# Autodesk Inventor assembly: 50
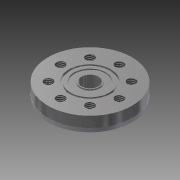
[picture p0: Inventor's stored thumbnail of the model, 180x180]
Saved by Autodesk Inventor 2013 (Build 170138000, 138)
## iProperties
Created: 2014-03-12
Part Number: 50
Document SubType Name: Assembly
Designer: andou
Author: andou
Title: Free-Horn
## Documents named in this file (5)
- C:\Users\andou\Documents\GitHub\Robotics-Project\design\RoboticsProject\project_4\Free_Horn.iam
- C:\Users\andou\Documents\GitHub\Robotics-Project\design\RoboticsProject\project_4\Bearing_Holder.ipt
- C:\Users\andou\Documents\GitHub\Robotics-Project\design\RoboticsProject\project_4\Generic Parts\Bearing.ipt
- C:\Users\andou\Documents\GitHub\Robotics-Project\design\RoboticsProject\project_4\Acetal_Washer.ipt
- C:\Users\andou\Documents\GitHub\Robotics-Project\design\RoboticsProject\project_4\Bearing_Washer.ipt
## Components (4 placed, 4 different names)
1. Bearing_Holder:1 — 挿入:1, 挿入:2
2. Bearing:1 — 挿入:1, 挿入:3
3. Acetal_Washer:1 — 挿入:2
4. Bearing_Washer:1 — 挿入:3
## Relationships (3: Insert 3)
- 挿入:1 [Insert]: Bearing_Holder:1 ↔ Bearing:1
- 挿入:2 [Insert]: Bearing_Holder:1 ↔ Acetal_Washer:1
- 挿入:3 [Insert]: Bearing:1 ↔ Bearing_Washer:1
